# Autodesk Inventor assembly: 50-J5
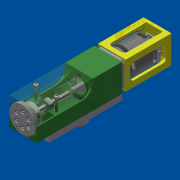
[picture p0: Inventor's stored thumbnail of the model, 180x180]
Saved by Autodesk Inventor 2018 (Build 220112000, 112)
## iProperties
Created: 2020-07-02
Part Number: 50-J5
Document SubType Name: Assembly
Designer: Bunny320
Author: Bunny320
## Documents named in this file (15)
- C:\Users\Bunny320\Desktop\sechs\4-CAD\50-J5.iam
- C:\Users\Bunny320\Desktop\sechs\4-CAD\motor unit 2820.iam
- C:\Users\Bunny320\Desktop\sechs\4-CAD\502-gearbox-housing.ipt
- C:\Users\Bunny320\Desktop\sechs\4-CAD\standardParts\W 606-2Z\W 606-2Z.iam
- C:\Users\Bunny320\Desktop\sechs\4-CAD\standardParts\61705-2RZ\W 61705-2RZ.iam
- C:\Users\Bunny320\Desktop\sechs\4-CAD\405-output disk.ipt
- C:\Users\Bunny320\Desktop\sechs\4-CAD\504-shaft.ipt
- C:\Users\Bunny320\Desktop\sechs\4-CAD\403-coupler dummy.ipt
- C:\Users\Bunny320\Desktop\sechs\4-CAD\standardParts\Pololu mounting hub\pololu-universal-aluminum-mounting-hub-for-6mm-shaft-m3-holes.ipt
- C:\Users\Bunny320\Desktop\sechs\4-CAD\501-flange.ipt
- C:\Users\Bunny320\Desktop\sechs\4-CAD\502-gearbox-housing-cap.ipt
- C:\Users\Bunny320\Documents\Inventor\Content Center Files\R2018\en-US\ISO 10642(2)\ISO 10642  - M3  x  12.ipt
- C:\Users\Bunny320\Documents\Inventor\Content Center Files\R2018\en-US\ISO 4762(1)\DIN EN ISO 4762 - M3 x 25.ipt
- C:\Users\Bunny320\Documents\Inventor\Content Center Files\R2018\en-US\ISO 4762(1)\DIN EN ISO 4762 - M3 x 12.ipt
- C:\Users\Bunny320\Documents\Inventor\Content Center Files\R2018\en-US\ISO 4762(1)\DIN EN ISO 4762 - M3 x 8.ipt
## Components (36 placed, 14 different names)
1. motor unit 2820:1 [sub-assembly] — Flush:1, Flush:2, Flush:3, Mate:1, Mate:2, Mate:3, Mate:9, Mate:10
2. 502-gearbox-housing:1 — Mate:1, Mate:2, Mate:3, Mate:4, Mate:5, Mate:6, Flush:4, Mate:13, Mate:14, Mate:15, Mate:16, Mate:17, Mate:18, Mate:19, Mate:20, Mate:21, Mate:22
3. W 606-2Z:1 [sub-assembly] — Mate:4, Mate:5
4. W 61705-2RZ:1 [sub-assembly] — Mate:6, Mate:7, Mate:8, Flush:4
5. 405-output disk:1 — Mate:7, Mate:8, Mate:12, Mate:55, Mate:56, Mate:57, Mate:58, Mate:59, Mate:60, Mate:61, Mate:62, Mate:63, Mate:64, Mate:65, Mate:66
6. 504-shaft:1 — Mate:9, Mate:11
7. 403-coupler dummy:1 — Mate:10
8. pololu-universal-aluminum-mounting-hub-for-6mm-shaft-m3-holes:1 — Mate:11, Mate:12
9. 501-flange:1 — Mate:13, Mate:14, Mate:15, Mate:27, Mate:28, Mate:29, Mate:30, Mate:31, Mate:32, Mate:33, Mate:34, Mate:35, Mate:36, Mate:37, Mate:38, Mate:39, Mate:40, Mate:41, Mate:42, Mate:43, Mate:44, Mate:45, Mate:46, Mate:47, Mate:48, Mate:49, Mate:50, Mate:51, Mate:52, Mate:53, Mate:54
10. 502-gearbox-housing-cap:1 — Mate:16, Mate:17, Mate:18, Mate:23, Mate:24, Mate:25, Mate:26
11. DIN EN ISO 10642 M3  x  12:1 — Mate:19
12. DIN EN ISO 10642 M3  x  12:2 — Mate:20
13. DIN EN ISO 10642 M3  x  12:3 — Mate:21
14. DIN EN ISO 10642 M3  x  12:4 — Mate:22
15. DIN EN ISO 4762 M3 x 25:1 — Mate:23, Mate:24
16. DIN EN ISO 4762 M3 x 25:2 — Mate:25, Mate:26
17. DIN EN ISO 4762 M3 x 12:1 — Mate:27, Mate:28
18. DIN EN ISO 4762 M3 x 12:2 — Mate:29, Mate:30
19. DIN EN ISO 4762 M3 x 12:3 — Mate:31, Mate:32
20. DIN EN ISO 4762 M3 x 12:4 — Mate:33, Mate:34
21. DIN EN ISO 4762 M3 x 12:5 — Mate:35, Mate:36
22. DIN EN ISO 4762 M3 x 12:6 — Mate:37, Mate:38
23. DIN EN ISO 4762 M3 x 8:1 — Mate:39, Mate:40
24. DIN EN ISO 4762 M3 x 8:2 — Mate:41, Mate:42
25. DIN EN ISO 4762 M3 x 8:3 — Mate:43, Mate:44
26. DIN EN ISO 4762 M3 x 8:4 — Mate:45, Mate:46
27. DIN EN ISO 4762 M3 x 8:5 — Mate:47, Mate:48
28. DIN EN ISO 4762 M3 x 8:6 — Mate:49, Mate:50
29. DIN EN ISO 4762 M3 x 8:7 — Mate:51, Mate:52
30. DIN EN ISO 4762 M3 x 8:8 — Mate:53, Mate:54
31. DIN EN ISO 4762 M3 x 12:7 — Mate:55, Mate:56
32. DIN EN ISO 4762 M3 x 12:8 — Mate:57, Mate:58
33. DIN EN ISO 4762 M3 x 12:9 — Mate:59, Mate:60
34. DIN EN ISO 4762 M3 x 12:10 — Mate:61, Mate:62
35. DIN EN ISO 4762 M3 x 12:11 — Mate:63, Mate:64
36. DIN EN ISO 4762 M3 x 12:12 — Mate:65, Mate:66
## Relationships (70: Mate 66, Flush 4)
- Flush:1: motor unit 2820:1
- Flush:2: motor unit 2820:1
- Flush:3: motor unit 2820:1
- Mate:1: motor unit 2820:1 ↔ 502-gearbox-housing:1
- Mate:2: motor unit 2820:1 ↔ 502-gearbox-housing:1
- Mate:3: motor unit 2820:1 ↔ 502-gearbox-housing:1
- Mate:4: 502-gearbox-housing:1 ↔ W 606-2Z:1
- Mate:5: 502-gearbox-housing:1 ↔ W 606-2Z:1
- Mate:6: 502-gearbox-housing:1 ↔ W 61705-2RZ:1
- Mate:7: W 61705-2RZ:1 ↔ 405-output disk:1
- Mate:8: W 61705-2RZ:1 ↔ 405-output disk:1
- Flush:4: 502-gearbox-housing:1 ↔ W 61705-2RZ:1
- Mate:9: motor unit 2820:1 ↔ 504-shaft:1
- Mate:10: motor unit 2820:1 ↔ 403-coupler dummy:1
- Mate:11: 504-shaft:1 ↔ pololu-universal-aluminum-mounting-hub-for-6mm-shaft-m3-holes:1
- Mate:12: 405-output disk:1 ↔ pololu-universal-aluminum-mounting-hub-for-6mm-shaft-m3-holes:1
- Mate:13: 502-gearbox-housing:1 ↔ 501-flange:1
- Mate:14: 502-gearbox-housing:1 ↔ 501-flange:1
- Mate:15: 502-gearbox-housing:1 ↔ 501-flange:1
- Mate:16: 502-gearbox-housing:1 ↔ 502-gearbox-housing-cap:1
- Mate:17: 502-gearbox-housing:1 ↔ 502-gearbox-housing-cap:1
- Mate:18: 502-gearbox-housing:1 ↔ 502-gearbox-housing-cap:1
- Mate:19: 502-gearbox-housing:1 ↔ DIN EN ISO 10642 M3  x  12:1
- Mate:20: 502-gearbox-housing:1 ↔ DIN EN ISO 10642 M3  x  12:2
- Mate:21: 502-gearbox-housing:1 ↔ DIN EN ISO 10642 M3  x  12:3
- Mate:22: 502-gearbox-housing:1 ↔ DIN EN ISO 10642 M3  x  12:4
- Mate:23: 502-gearbox-housing-cap:1 ↔ DIN EN ISO 4762 M3 x 25:1
- Mate:24: 502-gearbox-housing-cap:1 ↔ DIN EN ISO 4762 M3 x 25:1
- Mate:25: 502-gearbox-housing-cap:1 ↔ DIN EN ISO 4762 M3 x 25:2
- Mate:26: 502-gearbox-housing-cap:1 ↔ DIN EN ISO 4762 M3 x 25:2
- Mate:27: 501-flange:1 ↔ DIN EN ISO 4762 M3 x 12:1
- Mate:28: 501-flange:1 ↔ DIN EN ISO 4762 M3 x 12:1
- Mate:29: 501-flange:1 ↔ DIN EN ISO 4762 M3 x 12:2
- Mate:30: 501-flange:1 ↔ DIN EN ISO 4762 M3 x 12:2
- Mate:31: 501-flange:1 ↔ DIN EN ISO 4762 M3 x 12:3
- Mate:32: 501-flange:1 ↔ DIN EN ISO 4762 M3 x 12:3
- Mate:33: 501-flange:1 ↔ DIN EN ISO 4762 M3 x 12:4
- Mate:34: 501-flange:1 ↔ DIN EN ISO 4762 M3 x 12:4
- Mate:35: 501-flange:1 ↔ DIN EN ISO 4762 M3 x 12:5
- Mate:36: 501-flange:1 ↔ DIN EN ISO 4762 M3 x 12:5
- Mate:37: 501-flange:1 ↔ DIN EN ISO 4762 M3 x 12:6
- Mate:38: 501-flange:1 ↔ DIN EN ISO 4762 M3 x 12:6
- Mate:39: 501-flange:1 ↔ DIN EN ISO 4762 M3 x 8:1
- Mate:40: 501-flange:1 ↔ DIN EN ISO 4762 M3 x 8:1
- Mate:41: 501-flange:1 ↔ DIN EN ISO 4762 M3 x 8:2
- Mate:42: 501-flange:1 ↔ DIN EN ISO 4762 M3 x 8:2
- Mate:43: 501-flange:1 ↔ DIN EN ISO 4762 M3 x 8:3
- Mate:44: 501-flange:1 ↔ DIN EN ISO 4762 M3 x 8:3
- Mate:45: 501-flange:1 ↔ DIN EN ISO 4762 M3 x 8:4
- Mate:46: 501-flange:1 ↔ DIN EN ISO 4762 M3 x 8:4
- Mate:47: 501-flange:1 ↔ DIN EN ISO 4762 M3 x 8:5
- Mate:48: 501-flange:1 ↔ DIN EN ISO 4762 M3 x 8:5
- Mate:49: 501-flange:1 ↔ DIN EN ISO 4762 M3 x 8:6
- Mate:50: 501-flange:1 ↔ DIN EN ISO 4762 M3 x 8:6
- Mate:51: 501-flange:1 ↔ DIN EN ISO 4762 M3 x 8:7
- Mate:52: 501-flange:1 ↔ DIN EN ISO 4762 M3 x 8:7
- Mate:53: 501-flange:1 ↔ DIN EN ISO 4762 M3 x 8:8
- Mate:54: 501-flange:1 ↔ DIN EN ISO 4762 M3 x 8:8
- Mate:55: 405-output disk:1 ↔ DIN EN ISO 4762 M3 x 12:7
- Mate:56: 405-output disk:1 ↔ DIN EN ISO 4762 M3 x 12:7
- Mate:57: 405-output disk:1 ↔ DIN EN ISO 4762 M3 x 12:8
- Mate:58: 405-output disk:1 ↔ DIN EN ISO 4762 M3 x 12:8
- Mate:59: 405-output disk:1 ↔ DIN EN ISO 4762 M3 x 12:9
- Mate:60: 405-output disk:1 ↔ DIN EN ISO 4762 M3 x 12:9
- Mate:61: 405-output disk:1 ↔ DIN EN ISO 4762 M3 x 12:10
- Mate:62: 405-output disk:1 ↔ DIN EN ISO 4762 M3 x 12:10
- Mate:63: 405-output disk:1 ↔ DIN EN ISO 4762 M3 x 12:11
- Mate:64: 405-output disk:1 ↔ DIN EN ISO 4762 M3 x 12:11
- Mate:65: 405-output disk:1 ↔ DIN EN ISO 4762 M3 x 12:12
- Mate:66: 405-output disk:1 ↔ DIN EN ISO 4762 M3 x 12:12
